# Autodesk Inventor assembly: Assembly1
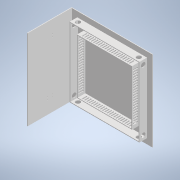
[picture p0: Inventor's stored thumbnail of the model, 180x180]
Saved by Autodesk Inventor 2020 (Build 240168000, 168)
## iProperties
Created: 2020-05-02
Part Number: Assembly1
Document SubType Name: Assembly
Designer: galaxy
Author: galaxy
## Documents named in this file (3)
- C:\Users\galaxy\Desktop\control box\Assembly1.iam
- C:\Users\galaxy\Desktop\control box\back.ipt
- C:\Users\galaxy\Desktop\control box\leftside.ipt
## Components (2 placed, 2 different names)
1. back:1 — Mate:1, Mate:2, Mate:3
2. leftside:1 — Mate:1, Mate:2, Mate:3
## Relationships (3: Mate 3)
- Mate:1: back:1 ↔ leftside:1
- Mate:2: back:1 ↔ leftside:1
- Mate:3: back:1 ↔ leftside:1
